# Autodesk Inventor assembly: st_bar_printasm
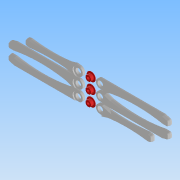
[picture p0: Inventor's stored thumbnail of the model, 180x180]
Saved by Autodesk Inventor 2021 (Build 250183000, 183)
## iProperties
Created: 2021-03-05
Part Number: st_bar_printasm
Document SubType Name: Assembly
Designer: kumagai
Author: kumagai
## Documents named in this file (5)
- X:\Develop\CAD\PlaRails\StoragePoint\st_bar_printasm.iam
- X:\Develop\CAD\PlaRails\StoragePoint\PocketPointBarPin.ipt
- X:\Develop\CAD\PlaRails\StoragePoint\PocketPointBar1.ipt
- X:\Develop\CAD\PlaRails\StoragePoint\PocketPointBar1_MIR.ipt
- X:\Develop\CAD\PlaRails\StoragePoint\PocketPointBar2.ipt
## Components (9 placed, 4 different names)
1. StoragePointBarPin:1
2. StoragePointBarPin:2
3. StoragePointBarPin:3
4. StoragePointBar2:1 — メイト:3, フラッシュ:3, メイト:6
5. StoragePointBar1_MIR:1 — メイト:2, フラッシュ:2, メイト:5
6. StoragePointBar1:1 — メイト:1, フラッシュ:1, メイト:4
7. StoragePointBar2:2
8. StoragePointBar1_MIR:2
9. StoragePointBar1:2
## Component patterns: (3 elements, first: StoragePointBarPin:1), (2 elements, first: StoragePointBar2:1 + StoragePointBar1_MIR:1 + StoragePointBar1:1)
## Relationships (9: Mate 6, Flush 3)
- メイト:1 [Mate]: StoragePointBar1:1
- メイト:2 [Mate] (10 mm): StoragePointBar1_MIR:1
- メイト:3 [Mate] (20 mm): StoragePointBar2:1
- フラッシュ:1 [Flush] (-10 mm): StoragePointBar1:1
- フラッシュ:2 [Flush] (10 mm): StoragePointBar1_MIR:1
- フラッシュ:3 [Flush] (10 mm): StoragePointBar2:1
- メイト:4 [Mate]: StoragePointBar1:1
- メイト:5 [Mate]: StoragePointBar1_MIR:1
- メイト:6 [Mate]: StoragePointBar2:1
